# Autodesk Inventor assembly: SoporteAluminio
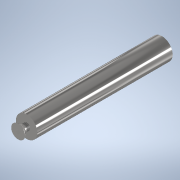
[picture p0: Inventor's stored thumbnail of the model, 180x180]
Saved by Autodesk Inventor 2020.3 (Build 243373010, 373A)
## iProperties
Created: 2020-11-14
Part Number: SoporteAluminio
Document SubType Name: Assembly
Designer: codig
Author: codig
## Documents named in this file (4)
- C:\Users\codig\Documents\GrabCAD\EscritorioV4\SoporteAluminio\SoporteAluminio.iam
- C:\Users\codig\Documents\GrabCAD\EscritorioV4\SoporteAluminio\Pieza1.ipt
- C:\Users\codig\Documents\Inventor\Content Center Files\R2020\es-ES\DIN 7991(2)\DIN 7991 - M8x16.ipt
- C:\Users\codig\Documents\GrabCAD\EscritorioV4\SoporteAluminio\Pieza3.ipt
## Components (3 placed, 3 different names)
1. Pieza1:1 — Cilíndrica:1, De rotación:1
2. DIN 7991 M8x16:1 — Cilíndrica:1
3. Pieza3:1 — De rotación:1
## Relationships (2: CylindricalJoint 1, RevoluteJoint 1)
- Cilíndrica:1 [CylindricalJoint]: Pieza1:1 ↔ DIN 7991 M8x16:1
- De rotación:1 [RevoluteJoint]: Pieza1:1 ↔ Pieza3:1
